# Autodesk Inventor assembly: ShooterPrototype-ver3-1111-2021
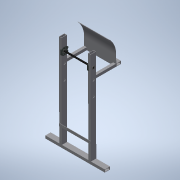
[picture p0: Inventor's stored thumbnail of the model, 180x180]
Saved by Autodesk Inventor 2021 (Build 250183000, 183)
## iProperties
Created: 2020-01-17
Part Number: ShooterPrototype-ver3-1111-2021
Document SubType Name: Assembly
Designer: JMHal
Author: JMHal
## Documents named in this file (10)
- F:\PHRC CADD 2021\PHRC CADD\2020 Infinite Recharge\Shooting\Assemblies\ShooterPrototype-ver3-1111-2021.iam
- F:\PHRC CADD 2021\PHRC CADD\2020 Infinite Recharge\Shooting\Parts\12in 2x1 Aluminum Block-ver1-1111-2019.ipt
- F:\PHRC CADD 2021\PHRC CADD\2020 Infinite Recharge\Shooting\Parts\16in 2x1 Aluminum Block-ver1-1111-2019.ipt
- F:\PHRC CADD 2021\PHRC CADD\2020 Infinite Recharge\Shooting\Parts\12in Aluminum Plate-ver-1-1111-2019.ipt
- F:\PHRC CADD 2021\PHRC CADD\Resources\Chassis Parts\0.5inThunderHexShaft(18in)-1111-2016.ipt
- F:\PHRC CADD 2021\PHRC CADD\2020 Infinite Recharge\Shooting\Parts\VersaBlock-ver1-1111-2019.ipt
- F:\PHRC CADD 2021\PHRC CADD\Resources\VEXpro Resources\Bearings\0.5inHexFlangedBearing(1.125inx0.313in)-1111-2016.ipt
- F:\PHRC CADD 2021\PHRC CADD\2020 Infinite Recharge\Shooting\Parts\ShooterBracketHorizontal.ver1-1111-2020.ipt
- F:\PHRC CADD 2021\PHRC CADD\2020 Infinite Recharge\Shooting\Parts\Hood.ver1-1111-2020.ipt
- F:\PHRC CADD 2021\PHRC CADD\2020 Infinite Recharge\Shooting\Parts\ShooterBracket.ver2-1111-2021.ipt
## Components (15 placed, 9 different names)
1. 12in 2x1 Aluminum Block-ver1-1111-2019:1 — Mate:22, Flush:5, Flush:6, Flush:7, Flush:18, Flush:20
2. 12in Aluminum Plate-ver-1-1111-2019:1 — Mate:12, Mate:13, Flush:2
3. 16in 2x1 Aluminum Block-ver1-1111-2019:3 — Mate:12, Mate:13, Cylindrical:2, Mate:16, Cylindrical:5, Mate:18, Angle:3, Flush:1, Flush:4, Flush:7, Symmetry:1, Mate:31, Flush:19, Angle:5
4. 16in 2x1 Aluminum Block-ver1-1111-2019:4 — Cylindrical:3, Mate:17, Cylindrical:6, Mate:19, Angle:4, Flush:2, Flush:4, Mate:22, Flush:5, Flush:6, Symmetry:1, Mate:30, Flush:17, Flush:25
5. 0.5inThunderHexShaft(18in)-1111-2016:1 — Cylindrical:7, Flush:1
6. 0.5inHexFlangedBearing(1.125inx0.313in)-1111-2016:1 — Cylindrical:2, Mate:16, Cylindrical:7, Mate:34
7. 0.5inHexFlangedBearing(1.125inx0.313in)-1111-2016:2 — Cylindrical:3, Mate:17
8. 0.5inHexFlangedBearing(1.125inx0.313in)-1111-2016:3 — Cylindrical:5, Mate:18, Rotational:3
9. VersaBlock-ver1-1111-2019:3 — Rotational:3, Angle:3
10. VersaBlock-ver1-1111-2019:4 — Rotational:4, Angle:4
11. 0.5inHexFlangedBearing(1.125inx0.313in)-1111-2016:4 — Cylindrical:6, Mate:19, Rotational:4
12. ShooterBracketHorizontal.ver1-1111-2020:1 — Mate:33, Flush:23, Flush:24
13. Hood.ver1-1111-2020:1 — Mate:32, Flush:21, Flush:22, Mate:33, Flush:23, Flush:24
14. ShooterBracket.ver2-1111-2021:1 — Mate:30, Flush:17, Flush:18, Mate:32, Flush:21, Flush:22
15. ShooterBracket.ver2-1111-2021:2 — Mate:31, Flush:19, Flush:20
## Relationships (39: Flush 16, Mate 12, CylindricalJoint 5, Angle 3, RevoluteJoint 2, Symmetry 1)
- Mate:12: 12in Aluminum Plate-ver-1-1111-2019:1 ↔ 16in 2x1 Aluminum Block-ver1-1111-2019:3
- Mate:13: 12in Aluminum Plate-ver-1-1111-2019:1 ↔ 16in 2x1 Aluminum Block-ver1-1111-2019:3
- Cylindrical:2: 16in 2x1 Aluminum Block-ver1-1111-2019:3 ↔ 0.5inHexFlangedBearing(1.125inx0.313in)-1111-2016:1
- Mate:16: 16in 2x1 Aluminum Block-ver1-1111-2019:3 ↔ 0.5inHexFlangedBearing(1.125inx0.313in)-1111-2016:1
- Cylindrical:3: 16in 2x1 Aluminum Block-ver1-1111-2019:4 ↔ 0.5inHexFlangedBearing(1.125inx0.313in)-1111-2016:2
- Mate:17: 16in 2x1 Aluminum Block-ver1-1111-2019:4 ↔ 0.5inHexFlangedBearing(1.125inx0.313in)-1111-2016:2
- Cylindrical:5: 16in 2x1 Aluminum Block-ver1-1111-2019:3 ↔ 0.5inHexFlangedBearing(1.125inx0.313in)-1111-2016:3
- Mate:18: 16in 2x1 Aluminum Block-ver1-1111-2019:3 ↔ 0.5inHexFlangedBearing(1.125inx0.313in)-1111-2016:3
- Rotational:3 [RevoluteJoint]: 0.5inHexFlangedBearing(1.125inx0.313in)-1111-2016:3 ↔ VersaBlock-ver1-1111-2019:3
- Angle:3 (0 deg): 16in 2x1 Aluminum Block-ver1-1111-2019:3 ↔ VersaBlock-ver1-1111-2019:3
- Cylindrical:6: 16in 2x1 Aluminum Block-ver1-1111-2019:4 ↔ 0.5inHexFlangedBearing(1.125inx0.313in)-1111-2016:4
- Mate:19: 16in 2x1 Aluminum Block-ver1-1111-2019:4 ↔ 0.5inHexFlangedBearing(1.125inx0.313in)-1111-2016:4
- Rotational:4 [RevoluteJoint]: VersaBlock-ver1-1111-2019:4 ↔ 0.5inHexFlangedBearing(1.125inx0.313in)-1111-2016:4
- Angle:4 (0 deg): 16in 2x1 Aluminum Block-ver1-1111-2019:4 ↔ VersaBlock-ver1-1111-2019:4
- Cylindrical:7: 0.5inThunderHexShaft(18in)-1111-2016:1 ↔ 0.5inHexFlangedBearing(1.125inx0.313in)-1111-2016:1
- Flush:1 (76.2 mm): 16in 2x1 Aluminum Block-ver1-1111-2019:3 ↔ 0.5inThunderHexShaft(18in)-1111-2016:1
- Flush:2: 12in Aluminum Plate-ver-1-1111-2019:1 ↔ 16in 2x1 Aluminum Block-ver1-1111-2019:4
- Flush:4: 16in 2x1 Aluminum Block-ver1-1111-2019:3 ↔ 16in 2x1 Aluminum Block-ver1-1111-2019:4
- Mate:22: 12in 2x1 Aluminum Block-ver1-1111-2019:1 ↔ 16in 2x1 Aluminum Block-ver1-1111-2019:4
- Flush:5: 12in 2x1 Aluminum Block-ver1-1111-2019:1 ↔ 16in 2x1 Aluminum Block-ver1-1111-2019:4
- Flush:6 (-133.35 mm): 12in 2x1 Aluminum Block-ver1-1111-2019:1 ↔ 16in 2x1 Aluminum Block-ver1-1111-2019:4
- Flush:7: 12in 2x1 Aluminum Block-ver1-1111-2019:1 ↔ 16in 2x1 Aluminum Block-ver1-1111-2019:3
- Symmetry:1: 16in 2x1 Aluminum Block-ver1-1111-2019:3 ↔ 16in 2x1 Aluminum Block-ver1-1111-2019:4
- Mate:30: 16in 2x1 Aluminum Block-ver1-1111-2019:4 ↔ ShooterBracket.ver2-1111-2021:1
- Flush:17: 16in 2x1 Aluminum Block-ver1-1111-2019:4 ↔ ShooterBracket.ver2-1111-2021:1
- Flush:18 (-692.15 mm): 12in 2x1 Aluminum Block-ver1-1111-2019:1 ↔ ShooterBracket.ver2-1111-2021:1
- Mate:31: 16in 2x1 Aluminum Block-ver1-1111-2019:3 ↔ ShooterBracket.ver2-1111-2021:2
- Flush:19: 16in 2x1 Aluminum Block-ver1-1111-2019:3 ↔ ShooterBracket.ver2-1111-2021:2
- Flush:20 (-692.15 mm): 12in 2x1 Aluminum Block-ver1-1111-2019:1 ↔ ShooterBracket.ver2-1111-2021:2
- Mate:32: Hood.ver1-1111-2020:1 ↔ ShooterBracket.ver2-1111-2021:1
- Flush:21: Hood.ver1-1111-2020:1 ↔ ShooterBracket.ver2-1111-2021:1
- Flush:22: Hood.ver1-1111-2020:1 ↔ ShooterBracket.ver2-1111-2021:1
- Mate:33: ShooterBracketHorizontal.ver1-1111-2020:1 ↔ Hood.ver1-1111-2020:1
- Flush:23: ShooterBracketHorizontal.ver1-1111-2020:1 ↔ Hood.ver1-1111-2020:1
- Flush:24: ShooterBracketHorizontal.ver1-1111-2020:1 ↔ Hood.ver1-1111-2020:1
- Flush:25 (1.778 mm): 16in 2x1 Aluminum Block-ver1-1111-2019:4
- Mate:34: 0.5inHexFlangedBearing(1.125inx0.313in)-1111-2016:1
- Angle:5 (0 deg): 16in 2x1 Aluminum Block-ver1-1111-2019:3
- Flush:26 (8.89 mm)
